# Autodesk Inventor assembly: Vision V2
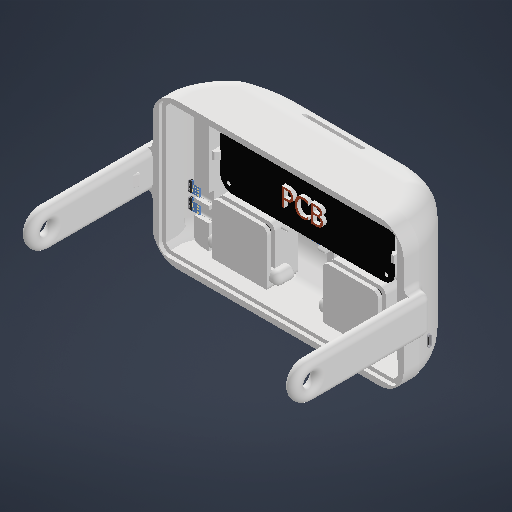
[picture p0: Inventor's stored thumbnail of the model, 512x512]
Saved by Autodesk Inventor 2025.1 (Build 291241020, 241B)
## iProperties
Created: 2024-04-29
Part Number: Vision V2
Document SubType Name: Assembly
Designer: techn
Author: techn
## Documents named in this file (11)
- C:\Users\techn\OneDrive\devMaxTrauma\3DModel\Vision V2.iam
- C:\Users\techn\OneDrive\devMaxTrauma\3DModel\VisionFrameV2.ipt
- C:\Users\techn\OneDrive\devMaxTrauma\3DModel\raspberry-pi-5-2.snapshot.7\RASPBERRY_PI_5\RASPBERRY_PI_5.iam
- C:\Users\techn\OneDrive\devMaxTrauma\3DModel\ultrasonic-sensors-hc-sr04-1.snapshot.2\HC-SR04.ipt
- C:\Users\techn\OneDrive\devMaxTrauma\3DModel\raspberry-pi-camera-module-v3-2.snapshot.4\Camera Moudule 3 v8\Camera Moudule 3 v8.iam
- C:\Users\techn\OneDrive\devMaxTrauma\3DModel\Raspberry Pi Display V1.1\Raspberry Pi Display V1.1.ipt
- C:\Users\techn\OneDrive\devMaxTrauma\3DModel\CoolingModule\CoolingModule.iam
- C:\Users\techn\OneDrive\devMaxTrauma\3DModel\usb-c-female-jrc-b008-1.snapshot.5\USB-C board JRC-B023\USB-C board JRC-B023.iam
- C:\Users\techn\OneDrive\devMaxTrauma\3DModel\PCB_Braket.ipt
- C:\Users\techn\OneDrive\devMaxTrauma\3DModel\PCB.ipt
- C:\Users\techn\OneDrive\devMaxTrauma\3DModel\LightSealGioV2.ipt
## Components (14 placed, 10 different names)
1. VisionFrameV2:1 — Rigid:1, Rigid:2, Rigid:3, Rigid:4, Rigid:6, Rigid:7, Rigid:9, Rigid:10, Rigid:11, Rigid:14
2. RASPBERRY_PI_5:1 [sub-assembly] — Rigid:1, Rigid:12
3. HC-SR04:1 — Rigid:2
4. Camera Moudule 3 v8:1 [sub-assembly] — Rigid:3
5. Camera Moudule 3 v8:2 [sub-assembly] — Rigid:4
6. CoolingModule:1 [sub-assembly] — Rigid:6
7. CoolingModule:2 [sub-assembly] — Rigid:7
8. USB-C board JRC-B023:1 [sub-assembly] — Rigid:9
9. USB-C board JRC-B023:2 [sub-assembly] — Rigid:11
10. USB-C board JRC-B023:3 [sub-assembly] — Rigid:10
11. PCB_Braket:1 — Rigid:12, Rigid:13
12. PCB:1 — Rigid:13
13. Raspberry Pi Display V1.1:1 — Rigid:14, Rigid:15
14. LightSealGioV2:1 — Rigid:15
## Relationships (13: WeldJoint 13)
- Rigid:1 [WeldJoint]: VisionFrameV2:1 ↔ RASPBERRY_PI_5:1
- Rigid:2 [WeldJoint]: VisionFrameV2:1 ↔ HC-SR04:1
- Rigid:3 [WeldJoint]: VisionFrameV2:1 ↔ Camera Moudule 3 v8:1
- Rigid:4 [WeldJoint]: VisionFrameV2:1 ↔ Camera Moudule 3 v8:2
- Rigid:6 [WeldJoint]: VisionFrameV2:1 ↔ CoolingModule:1
- Rigid:7 [WeldJoint]: VisionFrameV2:1 ↔ CoolingModule:2
- Rigid:9 [WeldJoint]: VisionFrameV2:1 ↔ USB-C board JRC-B023:1
- Rigid:10 [WeldJoint]: VisionFrameV2:1 ↔ USB-C board JRC-B023:3
- Rigid:11 [WeldJoint] (-2 mm): VisionFrameV2:1 ↔ USB-C board JRC-B023:2
- Rigid:12 [WeldJoint]: RASPBERRY_PI_5:1 ↔ PCB_Braket:1
- Rigid:13 [WeldJoint]: PCB_Braket:1 ↔ PCB:1
- Rigid:14 [WeldJoint]: VisionFrameV2:1 ↔ Raspberry Pi Display V1.1:1
- Rigid:15 [WeldJoint]: Raspberry Pi Display V1.1:1 ↔ LightSealGioV2:1
